# Autodesk Inventor assembly: Solar Panel
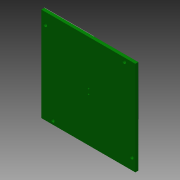
[picture p0: Inventor's stored thumbnail of the model, 180x180]
Saved by Autodesk Inventor 2015 SP1 (Build 190203100, 203)
## iProperties
Created: 2015-06-22
Part Number: Solar Panel
Document SubType Name: Assembly
Designer: Kartikye
Author: Kartikye
## Documents named in this file (3)
- C:\Users\Kartikye\Documents\GitHub\SASSat\Structure\Solar Panel.iam
- C:\Users\Kartikye\Documents\GitHub\SASSat\Structure\Solar Panel PCB.ipt
- C:\Users\Kartikye\Documents\GitHub\SASSat\Structure\Solar Cell.ipt
## Components (9 placed, 2 different names)
1. Solar Panel PCB:1 — Mate:1, Flush:1, Mate:2, Mate:3, Flush:2, Mate:4, Mate:5, Flush:3, Mate:6, Mate:7, Flush:4, Mate:8, Mate:9, Mate:10, Flush:5, Mate:11, Mate:12, Flush:6, Mate:13, Flush:7, Mate:14, Mate:15, Flush:8, Mate:16
2. Solar Cell:1 — Mate:1, Flush:1, Mate:2
3. Solar Cell:2 — Mate:9, Mate:10, Flush:5
4. Solar Cell:3 — Mate:3, Flush:2, Mate:4
5. Solar Cell:4 — Mate:11, Mate:12, Flush:6
6. Solar Cell:5 — Mate:5, Flush:3, Mate:6
7. Solar Cell:6 — Mate:13, Flush:7, Mate:14
8. Solar Cell:7 — Mate:7, Flush:4, Mate:8
9. Solar Cell:8 — Mate:15, Flush:8, Mate:16
## Relationships (24: Mate 16, Flush 8)
- Mate:1: Solar Panel PCB:1 ↔ Solar Cell:1
- Flush:1: Solar Panel PCB:1 ↔ Solar Cell:1
- Mate:2: Solar Panel PCB:1 ↔ Solar Cell:1
- Mate:3: Solar Panel PCB:1 ↔ Solar Cell:3
- Flush:2: Solar Panel PCB:1 ↔ Solar Cell:3
- Mate:4: Solar Panel PCB:1 ↔ Solar Cell:3
- Mate:5: Solar Panel PCB:1 ↔ Solar Cell:5
- Flush:3: Solar Panel PCB:1 ↔ Solar Cell:5
- Mate:6: Solar Panel PCB:1 ↔ Solar Cell:5
- Mate:7: Solar Panel PCB:1 ↔ Solar Cell:7
- Flush:4: Solar Panel PCB:1 ↔ Solar Cell:7
- Mate:8: Solar Panel PCB:1 ↔ Solar Cell:7
- Mate:9: Solar Panel PCB:1 ↔ Solar Cell:2
- Mate:10: Solar Panel PCB:1 ↔ Solar Cell:2
- Flush:5 (-12 mm): Solar Panel PCB:1 ↔ Solar Cell:2
- Mate:11: Solar Panel PCB:1 ↔ Solar Cell:4
- Mate:12: Solar Panel PCB:1 ↔ Solar Cell:4
- Flush:6 (12 mm): Solar Panel PCB:1 ↔ Solar Cell:4
- Mate:13: Solar Panel PCB:1 ↔ Solar Cell:6
- Flush:7 (12 mm): Solar Panel PCB:1 ↔ Solar Cell:6
- Mate:14: Solar Panel PCB:1 ↔ Solar Cell:6
- Mate:15: Solar Panel PCB:1 ↔ Solar Cell:8
- Flush:8 (12 mm): Solar Panel PCB:1 ↔ Solar Cell:8
- Mate:16: Solar Panel PCB:1 ↔ Solar Cell:8
